# Autodesk Inventor assembly: Top
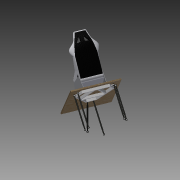
[picture p0: Inventor's stored thumbnail of the model, 180x180]
Saved by Autodesk Inventor 2015 (Build 190159000, 159)
## iProperties
Created: 2016-03-21
Part Number: Top
Document SubType Name: Assembly
Designer: Mac
Author: Mac
## Documents named in this file (5)
- C:\Users\Mac\Desktop\MotionBase\CAD\MotionBaseCAD\Top.iam
- C:\Users\Mac\Desktop\MotionBase\CAD\MotionBaseCAD\Platform.ipt
- C:\Users\Mac\Desktop\MotionBase\CAD\MotionBaseCAD\Rod.ipt
- C:\Users\Mac\Desktop\MotionBase\CAD\MotionBaseCAD\TopPlatform.ipt
- C:\Users\Mac\Desktop\MotionBase\CAD\MotionBaseCAD\Chair.iam
## Components (15 placed, 4 different names)
1. Platform:1 — Mate:7, Mate:8, Mate:9, Mate:10, Mate:11, Mate:12, Mate:13, Mate:14, Flush:7
2. Rod:7 — Mate:1, Flush:1, Mate:12
3. Rod:8 — Mate:1, Flush:1
4. Rod:9 — Mate:7
5. Rod:10
6. Rod:11 — Mate:11
7. Rod:12
8. Rod:13 — Mate:8
9. Rod:14
10. Rod:15 — Mate:10
11. Rod:16
12. Rod:17 — Mate:9
13. Rod:18
14. TopPlatform:1 — Mate:13, Mate:14, Flush:7, Mate:15, Flush:8
15. Chair:1 [sub-assembly] — Mate:15, Flush:8
## Relationships (23: Mate 15, Flush 8)
- Mate:1: Rod:7 ↔ Rod:8
- Flush:1: Rod:7 ↔ Rod:8
- [Mate]: Rod:9 ↔ Rod:10
- [Flush]: Rod:9 ↔ Rod:10
- [Mate]: Rod:11 ↔ Rod:12
- [Flush]: Rod:11 ↔ Rod:12
- [Mate]: Rod:13 ↔ Rod:14
- [Flush]: Rod:13 ↔ Rod:14
- [Mate]: Rod:15 ↔ Rod:16
- [Flush]: Rod:15 ↔ Rod:16
- [Mate]: Rod:17 ↔ Rod:18
- [Flush]: Rod:17 ↔ Rod:18
- Mate:7: Platform:1 ↔ Rod:9
- Mate:8: Platform:1 ↔ Rod:13
- Mate:9: Platform:1 ↔ Rod:17
- Mate:10: Platform:1 ↔ Rod:15
- Mate:11: Platform:1 ↔ Rod:11
- Mate:12: Platform:1 ↔ Rod:7
- Mate:13: Platform:1 ↔ TopPlatform:1
- Mate:14 (19.05 mm): Platform:1 ↔ TopPlatform:1
- Flush:7 (-76.2 mm): Platform:1 ↔ TopPlatform:1
- Mate:15: TopPlatform:1 ↔ Chair:1
- Flush:8 (152.4 mm): TopPlatform:1 ↔ Chair:1
## Named parameters: d2_d0 = 0 mm, d3_d1 = 0 mm, d4_d0 = 0 mm, d5_d1 = 0 mm, d6_d0 = 0 mm, d7_d1 = 0 mm, d8_d0 = 0 mm, d9_d1 = 0 mm, d10_d0 = 0 mm, d11_d1 = 0 mm
